# Autodesk Inventor assembly: Butterfly Drive Module
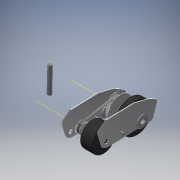
[picture p0: Inventor's stored thumbnail of the model, 180x180]
Saved by Autodesk Inventor 2019 (Build 230136000, 136)
## iProperties
Created: 2019-10-18
Part Number: Butterfly Drive Module
Document SubType Name: Assembly
Designer: admin
Author: admin
## Documents named in this file (8)
- C:\Users\Mark\Desktop\7738 Helion Engineering\7738-CAD-prep\Butterfly drive\Butterfly Drive Module.iam
- C:\Users\Mark\Desktop\7738 Helion Engineering\7738-CAD-prep\Butterfly drive\100mm Mecanum StandIn.ipt
- C:\Users\Mark\Desktop\7738 Helion Engineering\7738-CAD-prep\Butterfly drive\100mm Traction Wheel StandIn.ipt
- C:\Users\Mark\Desktop\7738 Helion Engineering\7738-CAD-prep\Butterfly drive\Butterfly Drive Module\Design Accelerator\Synchronous Belts Transmission3.iam
- C:\Users\Mark\Desktop\7738 Helion Engineering\7738-CAD-prep\Butterfly drive\Module Plate 1.ipt
- C:\Users\Mark\Desktop\7738 Helion Engineering\7738-CAD-prep\Butterfly drive\Connector.ipt
- C:\Users\Mark\Desktop\7738 Helion Engineering\7738-CAD-prep\Butterfly drive\F6004.ipt
- C:\Users\Mark\Desktop\7738 Helion Engineering\7738-CAD-prep\Butterfly drive\F6802.ipt
## Components (10 placed, 7 different names)
1. Connector:1 — Mate:34
2. 100mm Mecanum StandIn:1 — Flush:1, Mate:5, Angle:1, Mate:36, Mate:37
3. 100mm Traction Wheel StandIn:1 — Mate:4, Flush:1, Mate:6
4. Synchronous Belts Transmission:1 [sub-assembly] — Mate:5, Mate:6, Mate:35, Mate:37
5. Module Plate 1:1 — Mate:33, Flush:2, Flush:3, Mate:35, Mate:36, Insert:2, Insert:3
6. Module Plate 1:2 — Mate:33, Flush:2, Flush:3, Insert:1, Insert:4
7. F6804:1 — Insert:2
8. F6802:1 — Insert:4
9. F6804:2 — Insert:1
10. F6802:2 — Insert:3
## Relationships (16: Mate 8, Insert 4, Flush 3, Angle 1)
- Mate:4: 100mm Traction Wheel StandIn:1
- Flush:1 (10 mm): 100mm Mecanum StandIn:1 ↔ 100mm Traction Wheel StandIn:1
- Mate:5: 100mm Mecanum StandIn:1 ↔ Synchronous Belts Transmission:1
- Mate:6: 100mm Traction Wheel StandIn:1 ↔ Synchronous Belts Transmission:1
- Angle:1 (90 deg): 100mm Mecanum StandIn:1
- Mate:33 (105 mm): Module Plate 1:1 ↔ Module Plate 1:2
- Mate:34: Connector:1
- Flush:2: Module Plate 1:1 ↔ Module Plate 1:2
- Flush:3: Module Plate 1:1 ↔ Module Plate 1:2
- Mate:35: Synchronous Belts Transmission:1 ↔ Module Plate 1:1
- Mate:36 (4 mm): 100mm Mecanum StandIn:1 ↔ Module Plate 1:1
- Insert:1: Module Plate 1:2 ↔ F6804:2
- Insert:2: Module Plate 1:1 ↔ F6804:1
- Mate:37 (2 mm): 100mm Mecanum StandIn:1 ↔ Synchronous Belts Transmission:1
- Insert:3: Module Plate 1:1 ↔ F6802:2
- Insert:4: Module Plate 1:2 ↔ F6802:1
